# Autodesk Inventor assembly: BoronProbe_2026_non-bellows
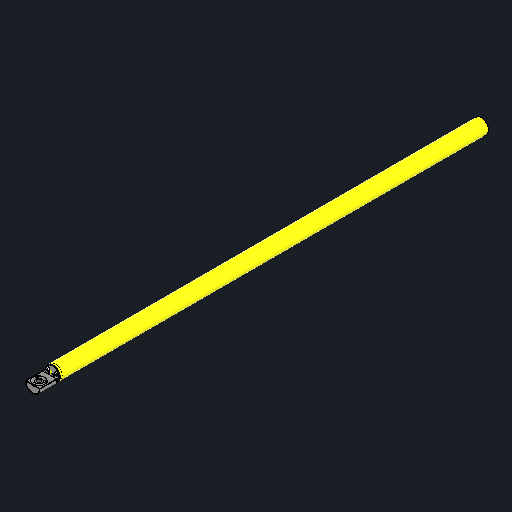
[picture p0: Inventor's stored thumbnail of the model, 512x512]
Saved by Autodesk Inventor 2027.1 (Build 311270010, 270A)
## iProperties
Created: 2026-05-08
Part Number: BoronProbe_2026_non-bellows
Document SubType Name: Assembly
Designer: zetsu
Author: zetsu
## Documents named in this file (17)
- C:\Users\queezz\Dropbox\Drawings\pihti-cad\BoronProbe_2026\BoronProbe_2026_non-bellows.iam
- C:\Users\queezz\Dropbox\Drawings\pihti-cad\BoronProbe_2026\parts\B_probehead_5.ipt
- C:\Users\queezz\Dropbox\Drawings\pihti-cad\BoronProbe_2026\parts\B_holder_sub_5.ipt
- C:\Users\queezz\Dropbox\Drawings\pihti-cad\BoronProbe_2026\parts\B_pipe_cylinder_5.ipt
- C:\Users\queezz\Dropbox\Drawings\pihti-cad\ContentCenter\Fastners\M3x6-BHCS.ipt
- C:\Users\queezz\Dropbox\Drawings\pihti-cad\ContentCenter\Ceramics\ceramic_bushing_M3-v1.ipt
- C:\Users\queezz\Dropbox\Drawings\pihti-cad\ContentCenter\Ceramics\ceramic_washer_M4_v1.ipt
- C:\Users\queezz\Dropbox\Drawings\pihti-cad\BoronProbe_2026\parts\B_shield_5.iam
- C:\Users\queezz\Dropbox\Drawings\pihti-cad\BoronProbe_2026\parts\ceramic_spacer_d3-13.ipt
- C:\Users\queezz\Dropbox\Drawings\pihti-cad\BoronProbe_2026\parts\ceramic_2-hole-spacer_d3-13.ipt
- C:\Users\queezz\Dropbox\Drawings\pihti-cad\BoronProbe_2026\parts\M2-4_screw.ipt
- C:\Users\queezz\Dropbox\Drawings\pihti-cad\BoronProbe_2026\parts\C25K22A4CU.iam
- C:\Users\queezz\Dropbox\Drawings\pihti-cad\BoronProbe_2026\parts\substrate.ipt
- C:\Users\queezz\Dropbox\Drawings\pihti-cad\ContentCenter\Fastners\M3-nut.ipt
- C:\Users\queezz\Dropbox\Drawings\pihti-cad\BoronProbe_2026\parts\B_holder_up_5.ipt
- C:\Users\queezz\Dropbox\Drawings\pihti-cad\BoronProbe_2026\parts\B_probe_pipe_5_for-non-bellows_1.ipt
- D:\repos\PIHTI\BoronProbe_2026\parts\ICF70-34-hole.ipt
## Components (31 placed, 16 different names)
1. B_probehead_5:1 — Mate:1, Mate:2, Mate:3, Mate:4, Mate:6, Mate:12, Mate:13, Mate:14, Mate:15, Mate:16, Mate:17, Mate:18, Mate:20, Mate:22, Mate:49, Mate:50, Mate:51, Mate:53, Flush:2, Mate:54, Flush:3, Mate:55, Flush:4
2. B_holder_sub_5:1 — Mate:1, Mate:2, Mate:3, Mate:5, Mate:7, Mate:76, Mate:77, Mate:78, Mate:79, Mate:80, Mate:81, Mate:82, Mate:83, Mate:86
3. Broached Hexagon Socket Button Head Cap Screw - Metric M3 x 0.5 x 6:1 — Mate:4, Mate:5
4. Broached Hexagon Socket Button Head Cap Screw - Metric M3 x 0.5 x 6:2 — Mate:6, Mate:7
5. Broached Hexagon Socket Button Head Cap Screw - Metric M3 x 0.5 x 6:5 — Mate:40, Mate:41
6. ceramic_bushing_M3-v1:1 — Mate:16, Mate:17, Mate:23, Mate:36, Mate:37
7. ceramic_bushing_M3-v1:2 — Mate:14, Mate:15, Mate:19, Mate:40, Mate:41
8. ceramic_bushing_M3-v1:3 — Mate:12, Mate:13, Mate:21, Mate:38, Mate:39
9. ceramic_washer_M4_v1:1 — Mate:20, Mate:21, Mate:43
10. ceramic_washer_M4_v1:2 — Mate:18, Mate:19, Mate:42
11. ceramic_washer_M4_v1:3 — Mate:22, Mate:23, Mate:44
12. Broached Hexagon Socket Button Head Cap Screw - Metric M3 x 0.5 x 6:6 — Mate:38, Mate:39
13. Broached Hexagon Socket Button Head Cap Screw - Metric M3 x 0.5 x 6:7 — Mate:36, Mate:37
14. B_pipe_cylinder_5:1 — Mate:42, Mate:43, Mate:44, Mate:93, Mate:94
15. B_shield_5:1 [sub-assembly] — Mate:49, Mate:50, Mate:51, Mate:56, Mate:57, Mate:58, Mate:59
16. ceramic_spacer_d3-13:1 — Mate:53, Flush:2
17. ceramic_spacer_d3-13:2 — Mate:54, Flush:3
18. ceramic_2-hole-spacer_d3-13:1 — Mate:55, Flush:4
19. M2-4_screw:1 — Mate:56, Mate:57
20. M2-4_screw:2 — Mate:58, Mate:59
21. C25K22A4CU:1 [sub-assembly]
22. substrate:1 — Mate:76, Mate:77, Mate:84
23. JIS B 1181 Style 1 - Metric A M3:1 — Mate:78, Mate:79
24. JIS B 1181 Style 1 - Metric A M3:2 — Mate:82, Mate:83
25. JIS B 1181 Style 1 - Metric A M3:3 — Mate:80, Mate:81, Mate:85
26. B_holder_up_5:1 — Mate:84, Mate:85, Mate:86, Mate:87, Mate:88, Mate:89, Mate:90, Mate:91, Mate:92
27. Broached Hexagon Socket Button Head Cap Screw - Metric M3 x 0.5 x 6:8 — Mate:87, Mate:88
28. Broached Hexagon Socket Button Head Cap Screw - Metric M3 x 0.5 x 6:9 — Mate:89, Mate:90
29. Broached Hexagon Socket Button Head Cap Screw - Metric M3 x 0.5 x 6:10 — Mate:91, Mate:92
30. B_probe_pipe_5_for-non-bellows_1:1 — Mate:93, Mate:94, Mate:95, Flush:5
31. ICF70-34-hole:1 — Mate:95, Flush:5
## Relationships (62: Mate 58, Flush 4)
- Mate:1: B_probehead_5:1 ↔ B_holder_sub_5:1
- Mate:2: B_probehead_5:1 ↔ B_holder_sub_5:1
- Mate:3: B_probehead_5:1 ↔ B_holder_sub_5:1
- Mate:4: B_probehead_5:1 ↔ Broached Hexagon Socket Button Head Cap Screw - Metric M3 x 0.5 x 6:1
- Mate:5: B_holder_sub_5:1 ↔ Broached Hexagon Socket Button Head Cap Screw - Metric M3 x 0.5 x 6:1
- Mate:6: B_probehead_5:1 ↔ Broached Hexagon Socket Button Head Cap Screw - Metric M3 x 0.5 x 6:2
- Mate:7: B_holder_sub_5:1 ↔ Broached Hexagon Socket Button Head Cap Screw - Metric M3 x 0.5 x 6:2
- Mate:12: B_probehead_5:1 ↔ ceramic_bushing_M3-v1:3
- Mate:13: B_probehead_5:1 ↔ ceramic_bushing_M3-v1:3
- Mate:14: B_probehead_5:1 ↔ ceramic_bushing_M3-v1:2
- Mate:15: B_probehead_5:1 ↔ ceramic_bushing_M3-v1:2
- Mate:16: B_probehead_5:1 ↔ ceramic_bushing_M3-v1:1
- Mate:17: B_probehead_5:1 ↔ ceramic_bushing_M3-v1:1
- Mate:18: B_probehead_5:1 ↔ ceramic_washer_M4_v1:2
- Mate:19: ceramic_bushing_M3-v1:2 ↔ ceramic_washer_M4_v1:2
- Mate:20: B_probehead_5:1 ↔ ceramic_washer_M4_v1:1
- Mate:21: ceramic_bushing_M3-v1:3 ↔ ceramic_washer_M4_v1:1
- Mate:22: B_probehead_5:1 ↔ ceramic_washer_M4_v1:3
- Mate:23: ceramic_bushing_M3-v1:1 ↔ ceramic_washer_M4_v1:3
- Mate:36: ceramic_bushing_M3-v1:1 ↔ Broached Hexagon Socket Button Head Cap Screw - Metric M3 x 0.5 x 6:7
- Mate:37: ceramic_bushing_M3-v1:1 ↔ Broached Hexagon Socket Button Head Cap Screw - Metric M3 x 0.5 x 6:7
- Mate:38: ceramic_bushing_M3-v1:3 ↔ Broached Hexagon Socket Button Head Cap Screw - Metric M3 x 0.5 x 6:6
- Mate:39: ceramic_bushing_M3-v1:3 ↔ Broached Hexagon Socket Button Head Cap Screw - Metric M3 x 0.5 x 6:6
- Mate:40: Broached Hexagon Socket Button Head Cap Screw - Metric M3 x 0.5 x 6:5 ↔ ceramic_bushing_M3-v1:2
- Mate:41: Broached Hexagon Socket Button Head Cap Screw - Metric M3 x 0.5 x 6:5 ↔ ceramic_bushing_M3-v1:2
- Mate:42: ceramic_washer_M4_v1:2 ↔ B_pipe_cylinder_5:1
- Mate:43: ceramic_washer_M4_v1:1 ↔ B_pipe_cylinder_5:1
- Mate:44: ceramic_washer_M4_v1:3 ↔ B_pipe_cylinder_5:1
- Mate:49: B_probehead_5:1 ↔ B_shield_5:1
- Mate:50: B_probehead_5:1 ↔ B_shield_5:1
- Mate:51: B_probehead_5:1 ↔ B_shield_5:1
- Mate:53: B_probehead_5:1 ↔ ceramic_spacer_d3-13:1
- Flush:2: B_probehead_5:1 ↔ ceramic_spacer_d3-13:1
- Mate:54: B_probehead_5:1 ↔ ceramic_spacer_d3-13:2
- Flush:3: B_probehead_5:1 ↔ ceramic_spacer_d3-13:2
- Mate:55: B_probehead_5:1 ↔ ceramic_2-hole-spacer_d3-13:1
- Flush:4: B_probehead_5:1 ↔ ceramic_2-hole-spacer_d3-13:1
- Mate:56: B_shield_5:1 ↔ M2-4_screw:1
- Mate:57: B_shield_5:1 ↔ M2-4_screw:1
- Mate:58: B_shield_5:1 ↔ M2-4_screw:2
- Mate:59: B_shield_5:1 ↔ M2-4_screw:2
- Mate:76: B_holder_sub_5:1 ↔ substrate:1
- Mate:77: B_holder_sub_5:1 ↔ substrate:1
- Mate:78: B_holder_sub_5:1 ↔ JIS B 1181 Style 1 - Metric A M3:1
- Mate:79: B_holder_sub_5:1 ↔ JIS B 1181 Style 1 - Metric A M3:1
- Mate:80: B_holder_sub_5:1 ↔ JIS B 1181 Style 1 - Metric A M3:3
- Mate:81: B_holder_sub_5:1 ↔ JIS B 1181 Style 1 - Metric A M3:3
- Mate:82: B_holder_sub_5:1 ↔ JIS B 1181 Style 1 - Metric A M3:2
- Mate:83: B_holder_sub_5:1 ↔ JIS B 1181 Style 1 - Metric A M3:2
- Mate:84: substrate:1 ↔ B_holder_up_5:1
- Mate:85: JIS B 1181 Style 1 - Metric A M3:3 ↔ B_holder_up_5:1
- Mate:86: B_holder_sub_5:1 ↔ B_holder_up_5:1
- Mate:87: B_holder_up_5:1 ↔ Broached Hexagon Socket Button Head Cap Screw - Metric M3 x 0.5 x 6:8
- Mate:88: B_holder_up_5:1 ↔ Broached Hexagon Socket Button Head Cap Screw - Metric M3 x 0.5 x 6:8
- Mate:89: B_holder_up_5:1 ↔ Broached Hexagon Socket Button Head Cap Screw - Metric M3 x 0.5 x 6:9
- Mate:90: B_holder_up_5:1 ↔ Broached Hexagon Socket Button Head Cap Screw - Metric M3 x 0.5 x 6:9
- Mate:91: B_holder_up_5:1 ↔ Broached Hexagon Socket Button Head Cap Screw - Metric M3 x 0.5 x 6:10
- Mate:92: B_holder_up_5:1 ↔ Broached Hexagon Socket Button Head Cap Screw - Metric M3 x 0.5 x 6:10
- Mate:93: B_pipe_cylinder_5:1 ↔ B_probe_pipe_5_for-non-bellows_1:1
- Mate:94: B_pipe_cylinder_5:1 ↔ B_probe_pipe_5_for-non-bellows_1:1
- Mate:95: B_probe_pipe_5_for-non-bellows_1:1 ↔ ICF70-34-hole:1
- Flush:5: B_probe_pipe_5_for-non-bellows_1:1 ↔ ICF70-34-hole:1
